# Autodesk Inventor assembly: DELL 1909Wf
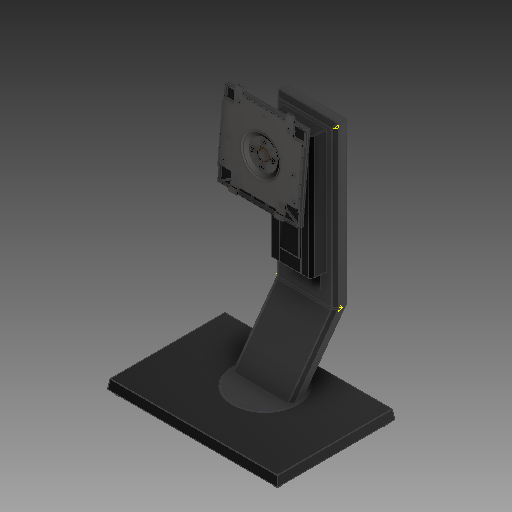
[picture p0: Inventor's stored thumbnail of the model, 512x512]
Saved by Autodesk Inventor 2017 SP1 (Build 210196100, 196)
## iProperties
Created: 2020-12-19
Part Number: DELL 1909Wf
Document SubType Name: Assembly
Designer: Napoleon
Author: Napoleon
## Documents named in this file (23)
- D:\PRYWATNE\PROJEKTY\POKÓJ\URZĄDZENIA PERYFERYJNE\DELL 1909Wf\PODSTAWA + STOJAK.iam
- D:\PRYWATNE\PROJEKTY\POKÓJ\URZĄDZENIA PERYFERYJNE\DELL 1909Wf\OBUDOWA PODSTAWY.ipt
- D:\PRYWATNE\PROJEKTY\POKÓJ\URZĄDZENIA PERYFERYJNE\DELL 1909Wf\PODSTAWA.ipt
- D:\PRYWATNE\PROJEKTY\POKÓJ\URZĄDZENIA PERYFERYJNE\DELL 1909Wf\PODUSZKA PODSTAWY.ipt
- D:\PRYWATNE\PROJEKTY\POKÓJ\URZĄDZENIA PERYFERYJNE\DELL 1909Wf\OBROTNICA.ipt
- D:\PRYWATNE\PROJEKTY\POKÓJ\URZĄDZENIA PERYFERYJNE\DELL 1909Wf\DOLNA PODSTAWA STOJAKA.ipt
- D:\PRYWATNE\PROJEKTY\POKÓJ\URZĄDZENIA PERYFERYJNE\DELL 1909Wf\TYLNA SZARA OBUDOWA STOJAKA.ipt
- D:\PRYWATNE\PROJEKTY\POKÓJ\URZĄDZENIA PERYFERYJNE\DELL 1909Wf\TYLNA CZARNA OBUDOWA STOJAKA.ipt
- D:\PRYWATNE\PROJEKTY\POKÓJ\URZĄDZENIA PERYFERYJNE\DELL 1909Wf\PRZEDNIA SZARA OBUDOWA STOJAKA.ipt
- D:\PRYWATNE\PROJEKTY\POKÓJ\URZĄDZENIA PERYFERYJNE\DELL 1909Wf\PRZEDNIA CZARNA OBUDOWA STOJAKA.ipt
- D:\PRYWATNE\PROJEKTY\POKÓJ\URZĄDZENIA PERYFERYJNE\DELL 1909Wf\ZAŚLEPKA PRZEDNIA GÓRNY CZARNEJ OBUDOWY STOJAKA.ipt
- D:\PRYWATNE\PROJEKTY\POKÓJ\URZĄDZENIA PERYFERYJNE\DELL 1909Wf\ZAŚLEPKA PRZEDNIA DOLNA CZARNEJ OBUDOWY STOJAKA.ipt
- D:\PRYWATNE\PROJEKTY\POKÓJ\URZĄDZENIA PERYFERYJNE\DELL 1909Wf\UCHWYT PIVOT.iam
- D:\PRYWATNE\PROJEKTY\POKÓJ\URZĄDZENIA PERYFERYJNE\DELL 1909Wf\PIVOT.iam
- D:\PRYWATNE\PROJEKTY\POKÓJ\URZĄDZENIA PERYFERYJNE\DELL 1909Wf\ŚRUBA + PODKŁADKI + NAKRĘTKA.iam
- C:\Users\Administrator\Documents\Inventor\Content Center Files\R2017\pl-PL\ANSI B18.16.3M(2)\ANSI B18.16.3M - Klasa właściwości 5 i 10 - Metryczny M5 x 0.8 Typ metalowy.ipt
- D:\PRYWATNE\PROJEKTY\POKÓJ\URZĄDZENIA PERYFERYJNE\DELL 1909Wf\OSŁONA MECHANIZMU PRZECHYLANIA MONITORA.ipt
- C:\Users\Administrator\Documents\Inventor\Content Center Files\R2017\pl-PL\ISO 7046-1(1)\DIN EN ISO 7046-1 - M3 x 4 - 4.8 - H.ipt
- D:\PRYWATNE\PROJEKTY\POKÓJ\URZĄDZENIA PERYFERYJNE\DELL 1909Wf\OSŁONA PIVOT.ipt
- D:\PRYWATNE\PROJEKTY\POKÓJ\URZĄDZENIA PERYFERYJNE\DELL 1909Wf\BLACHA CHWYTAJĄCA MONITOR.ipt
- D:\PRYWATNE\PROJEKTY\POKÓJ\URZĄDZENIA PERYFERYJNE\DELL 1909Wf\OSŁONA BLACHY CHWYTAJĄCEJ MONITOR.ipt
- C:\Users\Administrator\Documents\Inventor\Content Center Files\R2017\pl-PL\DIN 6798  A\DIN 6798 - A  4,3.ipt
- C:\Users\Administrator\Documents\Inventor\Content Center Files\R2017\pl-PL\ISO 7045(1)\DIN EN ISO 7045 - M4 x 5 - 4.8 - H.ipt
## Components (40 placed, 22 different names)
1. OBUDOWA PODSTAWY:1 — Równoległy:1
2. PODSTAWA:1 — Równoległy:1, Zestawiający:1, Sztywne:1, Sztywne:2, Sztywne:3, Sztywne:4, Sztywne:5, Sztywne:6, Sztywne:7
3. PODUSZKA PODSTAWY:1 — Zestawiający:1, Sztywne:5
4. PODUSZKA PODSTAWY:2 — Sztywne:1
5. PODUSZKA PODSTAWY:3 — Sztywne:2
6. PODUSZKA PODSTAWY:4 — Sztywne:3
7. PODUSZKA PODSTAWY:5 — Sztywne:6
8. PODUSZKA PODSTAWY:6 — Sztywne:4
9. OBROTNICA:1 — Sztywne:7, Obrotowe:1
10. DOLNA PODSTAWA STOJAKA:1 — Obrotowe:1, Sztywne:8
11. TYLNA SZARA OBUDOWA STOJAKA:1 — Sztywne:8, Zestawiający:2, Zestawiający:3, Zestawiający:4, Zestawiający:5, Równoległy:2, Równoległy:3
12. TYLNA CZARNA OBUDOWA STOJAKA:1 — Zestawiający:2, Zestawiający:3, Zestawiający:4, Równoległy:4, Zestawiający:7, Sztywne:9
13. PRZEDNIA SZARA OBUDOWA STOJAKA:1 — Zestawiający:5, Równoległy:2, Równoległy:3, Zestawiający:6
14. PRZEDNIA CZARNA OBUDOWA STOJAKA:1 — Zestawiający:6, Równoległy:4, Zestawiający:7, Zestawiający:8, Zestawiający:9
15. ZAŚLEPKA PRZEDNIA GÓRNY CZARNEJ OBUDOWY STOJAKA:1 — Zestawiający:8, Zestawiający:9, Równoległy:5, Równoległy:6, Równoległy:8, Równoległy:9
16. ZAŚLEPKA PRZEDNIA DOLNA CZARNEJ OBUDOWY STOJAKA:1 — Sztywne:9, Równoległy:5
17. UCHWYT PIVOT:1 [sub-assembly] — Równoległy:6, Równoległy:8, Równoległy:9, Obrotowe:2, Sztywne:10, Wstaw:1, Sztywne:11
18. PIVOT:1 [sub-assembly] — Obrotowe:2, Sztywne:12, Równoległy:10
19. ŚRUBA + PODKŁADKI + NAKRĘTKA:1 [sub-assembly] — Sztywne:10
20. Nakrętka samozabezpieczająca - Stal Metryczny Klasa właściwości 5 i 10 - Metryczny M5 x 0.8 Typ metalowy:1 — Wstaw:1
21. OSŁONA MECHANIZMU PRZECHYLANIA MONITORA:1 — Sztywne:11, Zestawiający:10, Zestawiający:11
22. DIN EN ISO 7046-1 H M3 x 4 - 4.8 - H:1 — Zestawiający:10
23. DIN EN ISO 7046-1 H M3 x 4 - 4.8 - H:2 — Zestawiający:11
24. OSŁONA PIVOT:1 — Sztywne:12, Zestawiający:18
25. BLACHA CHWYTAJĄCA MONITOR:1 — Równoległy:10, Zestawiający:12, Zestawiający:13, Zestawiający:14, Zestawiający:15, Zestawiający:16, Zestawiający:17, Wstaw:2, Wstaw:3, Wstaw:4, Wstaw:5
26. OSŁONA BLACHY CHWYTAJĄCEJ MONITOR:1 — Zestawiający:18
27. DIN EN ISO 7046-1 H M3 x 4 - 4.8 - H:3 — Zestawiający:12
28. DIN EN ISO 7046-1 H M3 x 4 - 4.8 - H:4 — Zestawiający:13
29. DIN EN ISO 7046-1 H M3 x 4 - 4.8 - H:5 — Zestawiający:14
30. DIN EN ISO 7046-1 H M3 x 4 - 4.8 - H:6 — Zestawiający:15
31. DIN EN ISO 7046-1 H M3 x 4 - 4.8 - H:7 — Zestawiający:16
32. DIN EN ISO 7046-1 H M3 x 4 - 4.8 - H:8 — Zestawiający:17
33. DIN 6798 A A  4,3:1 — Wstaw:2, Wstaw:6
34. DIN 6798 A A  4,3:2 — Wstaw:3, Wstaw:9
35. DIN 6798 A A  4,3:3 — Wstaw:4, Wstaw:7
36. DIN 6798 A A  4,3:4 — Wstaw:5, Wstaw:8
37. DIN EN ISO 7045 H M4 x 5 - 4.8 - H:1 — Wstaw:6
38. DIN EN ISO 7045 H M4 x 5 - 4.8 - H:2 — Wstaw:7
39. DIN EN ISO 7045 H M4 x 5 - 4.8 - H:3 — Wstaw:8
40. DIN EN ISO 7045 H M4 x 5 - 4.8 - H:4 — Wstaw:9
## Relationships (50: Mate 18, WeldJoint 12, Flush 9, Insert 9, RevoluteJoint 2)
- Równoległy:1 [Flush]: OBUDOWA PODSTAWY:1 ↔ PODSTAWA:1
- Zestawiający:1 [Mate]: PODSTAWA:1 ↔ PODUSZKA PODSTAWY:1
- Sztywne:1 [WeldJoint]: PODSTAWA:1 ↔ PODUSZKA PODSTAWY:2
- Sztywne:2 [WeldJoint]: PODSTAWA:1 ↔ PODUSZKA PODSTAWY:3
- Sztywne:3 [WeldJoint]: PODSTAWA:1 ↔ PODUSZKA PODSTAWY:4
- Sztywne:4 [WeldJoint]: PODSTAWA:1 ↔ PODUSZKA PODSTAWY:6
- Sztywne:5 [WeldJoint]: PODSTAWA:1 ↔ PODUSZKA PODSTAWY:1
- Sztywne:6 [WeldJoint]: PODSTAWA:1 ↔ PODUSZKA PODSTAWY:5
- Sztywne:7 [WeldJoint]: PODSTAWA:1 ↔ OBROTNICA:1
- Obrotowe:1 [RevoluteJoint]: OBROTNICA:1 ↔ DOLNA PODSTAWA STOJAKA:1
- Sztywne:8 [WeldJoint]: DOLNA PODSTAWA STOJAKA:1 ↔ TYLNA SZARA OBUDOWA STOJAKA:1
- Zestawiający:2 [Mate]: TYLNA SZARA OBUDOWA STOJAKA:1 ↔ TYLNA CZARNA OBUDOWA STOJAKA:1
- Zestawiający:3 [Mate]: TYLNA SZARA OBUDOWA STOJAKA:1 ↔ TYLNA CZARNA OBUDOWA STOJAKA:1
- Zestawiający:4 [Mate] (-10 mm): TYLNA SZARA OBUDOWA STOJAKA:1 ↔ TYLNA CZARNA OBUDOWA STOJAKA:1
- Zestawiający:5 [Mate]: TYLNA SZARA OBUDOWA STOJAKA:1 ↔ PRZEDNIA SZARA OBUDOWA STOJAKA:1
- Równoległy:2 [Flush]: TYLNA SZARA OBUDOWA STOJAKA:1 ↔ PRZEDNIA SZARA OBUDOWA STOJAKA:1
- Równoległy:3 [Flush]: TYLNA SZARA OBUDOWA STOJAKA:1 ↔ PRZEDNIA SZARA OBUDOWA STOJAKA:1
- Zestawiający:6 [Mate]: PRZEDNIA SZARA OBUDOWA STOJAKA:1 ↔ PRZEDNIA CZARNA OBUDOWA STOJAKA:1
- Równoległy:4 [Flush]: TYLNA CZARNA OBUDOWA STOJAKA:1 ↔ PRZEDNIA CZARNA OBUDOWA STOJAKA:1
- Zestawiający:7 [Mate]: TYLNA CZARNA OBUDOWA STOJAKA:1 ↔ PRZEDNIA CZARNA OBUDOWA STOJAKA:1
- Sztywne:9 [WeldJoint]: TYLNA CZARNA OBUDOWA STOJAKA:1 ↔ ZAŚLEPKA PRZEDNIA DOLNA CZARNEJ OBUDOWY STOJAKA:1
- Zestawiający:8 [Mate] (3.989 mm): PRZEDNIA CZARNA OBUDOWA STOJAKA:1 ↔ ZAŚLEPKA PRZEDNIA GÓRNY CZARNEJ OBUDOWY STOJAKA:1
- Zestawiający:9 [Mate] (0.5 mm): PRZEDNIA CZARNA OBUDOWA STOJAKA:1 ↔ ZAŚLEPKA PRZEDNIA GÓRNY CZARNEJ OBUDOWY STOJAKA:1
- Równoległy:5 [Flush]: ZAŚLEPKA PRZEDNIA GÓRNY CZARNEJ OBUDOWY STOJAKA:1 ↔ ZAŚLEPKA PRZEDNIA DOLNA CZARNEJ OBUDOWY STOJAKA:1
- Równoległy:6 [Flush] (2.55 mm): ZAŚLEPKA PRZEDNIA GÓRNY CZARNEJ OBUDOWY STOJAKA:1 ↔ UCHWYT PIVOT:1
- Równoległy:8 [Flush] (1.675 mm): ZAŚLEPKA PRZEDNIA GÓRNY CZARNEJ OBUDOWY STOJAKA:1 ↔ UCHWYT PIVOT:1
- Równoległy:9 [Flush] (6 mm): ZAŚLEPKA PRZEDNIA GÓRNY CZARNEJ OBUDOWY STOJAKA:1 ↔ UCHWYT PIVOT:1
- Obrotowe:2 [RevoluteJoint]: UCHWYT PIVOT:1 ↔ PIVOT:1
- Sztywne:10 [WeldJoint]: UCHWYT PIVOT:1 ↔ ŚRUBA + PODKŁADKI + NAKRĘTKA:1
- Wstaw:1 [Insert]: UCHWYT PIVOT:1 ↔ Nakrętka samozabezpieczająca - Stal Metryczny Klasa właściwości 5 i 10 - Metryczny M5 x 0.8 Typ metalowy:1
- Sztywne:11 [WeldJoint]: UCHWYT PIVOT:1 ↔ OSŁONA MECHANIZMU PRZECHYLANIA MONITORA:1
- Zestawiający:10 [Mate]: OSŁONA MECHANIZMU PRZECHYLANIA MONITORA:1 ↔ DIN EN ISO 7046-1 H M3 x 4 - 4.8 - H:1
- Zestawiający:11 [Mate]: OSŁONA MECHANIZMU PRZECHYLANIA MONITORA:1 ↔ DIN EN ISO 7046-1 H M3 x 4 - 4.8 - H:2
- Sztywne:12 [WeldJoint]: PIVOT:1 ↔ OSŁONA PIVOT:1
- Równoległy:10 [Flush]: PIVOT:1 ↔ BLACHA CHWYTAJĄCA MONITOR:1
- Zestawiający:12 [Mate]: BLACHA CHWYTAJĄCA MONITOR:1 ↔ DIN EN ISO 7046-1 H M3 x 4 - 4.8 - H:3
- Zestawiający:13 [Mate]: BLACHA CHWYTAJĄCA MONITOR:1 ↔ DIN EN ISO 7046-1 H M3 x 4 - 4.8 - H:4
- Zestawiający:14 [Mate]: BLACHA CHWYTAJĄCA MONITOR:1 ↔ DIN EN ISO 7046-1 H M3 x 4 - 4.8 - H:5
- Zestawiający:15 [Mate]: BLACHA CHWYTAJĄCA MONITOR:1 ↔ DIN EN ISO 7046-1 H M3 x 4 - 4.8 - H:6
- Zestawiający:16 [Mate]: BLACHA CHWYTAJĄCA MONITOR:1 ↔ DIN EN ISO 7046-1 H M3 x 4 - 4.8 - H:7
- Zestawiający:17 [Mate]: BLACHA CHWYTAJĄCA MONITOR:1 ↔ DIN EN ISO 7046-1 H M3 x 4 - 4.8 - H:8
- Wstaw:2 [Insert]: BLACHA CHWYTAJĄCA MONITOR:1 ↔ DIN 6798 A A  4,3:1
- Wstaw:3 [Insert]: BLACHA CHWYTAJĄCA MONITOR:1 ↔ DIN 6798 A A  4,3:2
- Wstaw:4 [Insert]: BLACHA CHWYTAJĄCA MONITOR:1 ↔ DIN 6798 A A  4,3:3
- Wstaw:5 [Insert]: BLACHA CHWYTAJĄCA MONITOR:1 ↔ DIN 6798 A A  4,3:4
- Wstaw:6 [Insert]: DIN 6798 A A  4,3:1 ↔ DIN EN ISO 7045 H M4 x 5 - 4.8 - H:1
- Wstaw:7 [Insert]: DIN 6798 A A  4,3:3 ↔ DIN EN ISO 7045 H M4 x 5 - 4.8 - H:2
- Wstaw:8 [Insert]: DIN 6798 A A  4,3:4 ↔ DIN EN ISO 7045 H M4 x 5 - 4.8 - H:3
- Wstaw:9 [Insert]: DIN 6798 A A  4,3:2 ↔ DIN EN ISO 7045 H M4 x 5 - 4.8 - H:4
- Zestawiający:18 [Mate]: OSŁONA PIVOT:1 ↔ OSŁONA BLACHY CHWYTAJĄCEJ MONITOR:1
